# Autodesk Inventor assembly: X_rail_Assembly_Rev3
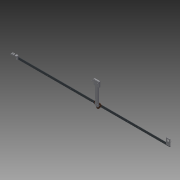
[picture p0: Inventor's stored thumbnail of the model, 180x180]
Saved by Autodesk Inventor 2015 (Build 190159000, 159)
## iProperties
Created: 2017-01-08
Part Number: X_rail_Assembly_Rev3
Document SubType Name: Assembly
Designer: Guy
Author: Guy
## Documents named in this file (12)
- C:\Users\Ernest\Documents\Capstone-Project\doc\CAD\LowLevel_Rev3\X_rail_Assembly_Rev3.iam
- C:\Users\Ernest\Documents\Capstone-Project\doc\CAD\LowLevel_Rev3\X_Rai-SquareBar-Rev3.ipt
- C:\Users\Ernest\Documents\Capstone-Project\doc\CAD\LowLevel_Rev3\XY_Wheel-SquareBar-Rev3.ipt
- C:\Users\Ernest\Documents\Capstone-Project\doc\CAD\LowLevel_Rev3\Arm-SquareBar-Rev3.ipt
- C:\Users\Ernest\Documents\Capstone-Project\doc\CAD\Nuts and Bolts\3-16in_1 1-4in_Bolt.ipt
- C:\Users\Ernest\Documents\Capstone-Project\doc\CAD\Nuts and Bolts\3-16in_7-16in_washer(num8).ipt
- C:\Users\Ernest\Documents\Capstone-Project\doc\CAD\Nuts and Bolts\3-16in_1-16in_nut(num2).ipt
- C:\Users\Ernest\Documents\Capstone-Project\doc\CAD\Stepper Motor\NEMA 23\NEMA 23 Holder.ipt
- C:\Users\Ernest\Documents\Capstone-Project\doc\CAD\LowLevel_Rev3\X_Rail_Belt_Pulley_Connector(2).ipt
- C:\Users\Ernest\Documents\Capstone-Project\doc\CAD\LowLevel_Rev3\X_Rail_Belt_Pulley_Connector.ipt
- C:\Users\Ernest\Documents\Capstone-Project\doc\CAD\LowLevel_Rev3\Arm_Base-SquareBar-Rev3-2.ipt
- C:\Users\Ernest\Documents\Capstone-Project\doc\CAD\Nuts and Bolts\L-Bracket.ipt
## Components (45 placed, 11 different names)
1. X_Rai-SquareBar-Rev3:1 — Tangent:3, Mate:3, Tangent:4, Tangent:5, Mate:88, Mate:133, Angle:2, Mate:174, Mate:175, Mate:176, Mate:177
2. XY_Wheel-SquareBar-Rev3:1 — Tangent:3, Mate:3, Flush:1, Mate:75, Mate:77, Mate:78
3. Arm-SquareBar-Rev3:1 — Mate:28, Mate:29, Mate:30, Mate:31, Mate:123, Mate:124, Mate:125, Mate:142, Mate:153, Angle:2, Mate:168, Mate:169, Mate:170, Mate:171, Mate:172, Mate:173
4. XY_Wheel-SquareBar-Rev3:2 — Tangent:4, Flush:2, Mate:68, Mate:69, Mate:118
5. XY_Wheel-SquareBar-Rev3:3 — Tangent:5, Flush:1, Flush:2, Mate:51, Mate:55, Mate:116
6. 3-16in_1 1-4in_Bolt:1 — Mate:40, Mate:41, Mate:142, Mate:156, Mate:157
7. 3-16in_7-16in_washer(num8):1 — Mate:29, Mate:32, Mate:36
8. 3-16in_7-16in_washer(num8):2 — Mate:28, Mate:33, Mate:38
9. 3-16in_7-16in_washer(num8):3 — Mate:30, Mate:35, Mate:40
10. 3-16in_7-16in_washer(num8):4 — Mate:31, Mate:34, Mate:42
11. 3-16in_1 1-4in_Bolt:2 — Mate:36, Mate:37, Mate:125, Mate:161
12. 3-16in_1 1-4in_Bolt:3 — Mate:42, Mate:43, Mate:123, Mate:154, Mate:160
13. 3-16in_1 1-4in_Bolt:4 — Mate:38, Mate:39, Mate:124, Mate:158, Mate:159
14. 3-16in_1-16in_nut(num2):1 — Mate:35, Mate:41
15. 3-16in_1-16in_nut(num2):2 — Mate:34, Mate:43, Mate:154
16. 3-16in_1-16in_nut(num2):3 — Mate:33, Mate:39
17. 3-16in_1-16in_nut(num2):4 — Mate:32, Mate:37
18. 3-16in_1 1-4in_Bolt:5 — Mate:46, Mate:48, Mate:49, Mate:52, Mate:53, Mate:116, Flush:4, Mate:146, Mate:149
19. 3-16in_1 1-4in_Bolt:6 — Mate:60, Mate:61, Mate:62, Mate:63, Mate:64, Mate:118, Mate:145, Mate:165
20. 3-16in_1 1-4in_Bolt:7 — Mate:70, Mate:71, Mate:72, Mate:73, Mate:74, Mate:75, Mate:164
21. 3-16in_1-16in_nut(num2):5 — Mate:46, Mate:148, Mate:149
22. 3-16in_1-16in_nut(num2):6 — Mate:48, Mate:50
23. 3-16in_1-16in_nut(num2):7 — Mate:53, Mate:54, Flush:4
24. 3-16in_7-16in_washer(num8):5 — Mate:49, Mate:50, Mate:55
25. 3-16in_7-16in_washer(num8):6 — Mate:51, Mate:52, Mate:54
26. 3-16in_7-16in_washer(num8):7 — Mate:56, Mate:63, Mate:69
27. 3-16in_7-16in_washer(num8):8 — Mate:57, Mate:61, Mate:68
28. 3-16in_7-16in_washer(num8):9 — Mate:58, Mate:73, Mate:78
29. 3-16in_7-16in_washer(num8):10 — Mate:59, Mate:71, Mate:77
30. 3-16in_1-16in_nut(num2):8 — Mate:56, Mate:64
31. 3-16in_1-16in_nut(num2):9 — Mate:57, Mate:62
32. 3-16in_1-16in_nut(num2):10 — Mate:60, Mate:147, Mate:165
33. 3-16in_1-16in_nut(num2):11 — Mate:58, Mate:74
34. 3-16in_1-16in_nut(num2):12 — Mate:59, Mate:72
35. 3-16in_1-16in_nut(num2):13 — Mate:70, Mate:163, Mate:164
36. NEMA 23 Holder:1 — Mate:88, Mate:106, Mate:107, Mate:141, Mate:174, Mate:175
37. XY_Wheel-SquareBar-Rev3:4 — Mate:93, Mate:140
38. 3-16in_1 1-4in_Bolt:8 — Mate:93, Mate:136, Mate:137
39. 3-16in_1 1-4in_Bolt:9 — Mate:106, Mate:107, Mate:109
40. 3-16in_1-16in_nut(num2):17 — Mate:109, Mate:141
41. X_Rail_Belt_Pulley_Connector(2):1 — Mate:136, Mate:137, Mate:138, Mate:139, Angle:1, Mate:140
42. X_Rail_Belt_Pulley_Connector:1 — Mate:133, Mate:138, Mate:139, Angle:1, Mate:176, Mate:177
43. Arm_Base-SquareBar-Rev3-2:1 — Mate:145, Mate:146, Mate:147, Mate:148, Mate:153, Mate:156, Mate:157, Mate:158, Mate:159, Mate:160, Mate:161, Mate:163
44. L-Bracket:1 — Mate:171, Mate:172, Mate:173
45. L-Bracket:2 — Mate:168, Mate:169, Mate:170
## Relationships (97: Mate 89, Tangent 3, Flush 3, Angle 2)
- Tangent:3: X_Rai-SquareBar-Rev3:1 ↔ XY_Wheel-SquareBar-Rev3:1
- Mate:3 (0.075 mm): X_Rai-SquareBar-Rev3:1 ↔ XY_Wheel-SquareBar-Rev3:1
- Tangent:4: X_Rai-SquareBar-Rev3:1 ↔ XY_Wheel-SquareBar-Rev3:2
- Tangent:5: X_Rai-SquareBar-Rev3:1 ↔ XY_Wheel-SquareBar-Rev3:3
- Flush:1: XY_Wheel-SquareBar-Rev3:1 ↔ XY_Wheel-SquareBar-Rev3:3
- Flush:2: XY_Wheel-SquareBar-Rev3:2 ↔ XY_Wheel-SquareBar-Rev3:3
- Mate:28: Arm-SquareBar-Rev3:1 ↔ 3-16in_7-16in_washer(num8):2
- Mate:29: Arm-SquareBar-Rev3:1 ↔ 3-16in_7-16in_washer(num8):1
- Mate:30: Arm-SquareBar-Rev3:1 ↔ 3-16in_7-16in_washer(num8):3
- Mate:31: Arm-SquareBar-Rev3:1 ↔ 3-16in_7-16in_washer(num8):4
- Mate:32: 3-16in_7-16in_washer(num8):1 ↔ 3-16in_1-16in_nut(num2):4
- Mate:33: 3-16in_7-16in_washer(num8):2 ↔ 3-16in_1-16in_nut(num2):3
- Mate:34: 3-16in_7-16in_washer(num8):4 ↔ 3-16in_1-16in_nut(num2):2
- Mate:35: 3-16in_7-16in_washer(num8):3 ↔ 3-16in_1-16in_nut(num2):1
- Mate:36: 3-16in_7-16in_washer(num8):1 ↔ 3-16in_1 1-4in_Bolt:2
- Mate:37: 3-16in_1 1-4in_Bolt:2 ↔ 3-16in_1-16in_nut(num2):4
- Mate:38: 3-16in_7-16in_washer(num8):2 ↔ 3-16in_1 1-4in_Bolt:4
- Mate:39: 3-16in_1 1-4in_Bolt:4 ↔ 3-16in_1-16in_nut(num2):3
- Mate:40: 3-16in_1 1-4in_Bolt:1 ↔ 3-16in_7-16in_washer(num8):3
- Mate:41: 3-16in_1 1-4in_Bolt:1 ↔ 3-16in_1-16in_nut(num2):1
- Mate:42: 3-16in_7-16in_washer(num8):4 ↔ 3-16in_1 1-4in_Bolt:3
- Mate:43: 3-16in_1 1-4in_Bolt:3 ↔ 3-16in_1-16in_nut(num2):2
- Mate:46: 3-16in_1 1-4in_Bolt:5 ↔ 3-16in_1-16in_nut(num2):5
- Mate:48: 3-16in_1 1-4in_Bolt:5 ↔ 3-16in_1-16in_nut(num2):6
- Mate:49: 3-16in_1 1-4in_Bolt:5 ↔ 3-16in_7-16in_washer(num8):5
- Mate:50: 3-16in_1-16in_nut(num2):6 ↔ 3-16in_7-16in_washer(num8):5
- Mate:51: XY_Wheel-SquareBar-Rev3:3 ↔ 3-16in_7-16in_washer(num8):6
- Mate:52: 3-16in_1 1-4in_Bolt:5 ↔ 3-16in_7-16in_washer(num8):6
- Mate:53: 3-16in_1 1-4in_Bolt:5 ↔ 3-16in_1-16in_nut(num2):7
- Mate:54: 3-16in_1-16in_nut(num2):7 ↔ 3-16in_7-16in_washer(num8):6
- Mate:55: XY_Wheel-SquareBar-Rev3:3 ↔ 3-16in_7-16in_washer(num8):5
- Mate:56: 3-16in_7-16in_washer(num8):7 ↔ 3-16in_1-16in_nut(num2):8
- Mate:57: 3-16in_7-16in_washer(num8):8 ↔ 3-16in_1-16in_nut(num2):9
- Mate:58: 3-16in_7-16in_washer(num8):9 ↔ 3-16in_1-16in_nut(num2):11
- Mate:59: 3-16in_7-16in_washer(num8):10 ↔ 3-16in_1-16in_nut(num2):12
- Mate:60: 3-16in_1 1-4in_Bolt:6 ↔ 3-16in_1-16in_nut(num2):10
- Mate:61: 3-16in_1 1-4in_Bolt:6 ↔ 3-16in_7-16in_washer(num8):8
- Mate:62: 3-16in_1 1-4in_Bolt:6 ↔ 3-16in_1-16in_nut(num2):9
- Mate:63: 3-16in_1 1-4in_Bolt:6 ↔ 3-16in_7-16in_washer(num8):7
- Mate:64: 3-16in_1 1-4in_Bolt:6 ↔ 3-16in_1-16in_nut(num2):8
- Mate:68: XY_Wheel-SquareBar-Rev3:2 ↔ 3-16in_7-16in_washer(num8):8
- Mate:69: XY_Wheel-SquareBar-Rev3:2 ↔ 3-16in_7-16in_washer(num8):7
- Mate:70: 3-16in_1 1-4in_Bolt:7 ↔ 3-16in_1-16in_nut(num2):13
- Mate:71: 3-16in_1 1-4in_Bolt:7 ↔ 3-16in_7-16in_washer(num8):10
- Mate:72: 3-16in_1 1-4in_Bolt:7 ↔ 3-16in_1-16in_nut(num2):12
- Mate:73: 3-16in_1 1-4in_Bolt:7 ↔ 3-16in_7-16in_washer(num8):9
- Mate:74: 3-16in_1 1-4in_Bolt:7 ↔ 3-16in_1-16in_nut(num2):11
- Mate:75: XY_Wheel-SquareBar-Rev3:1 ↔ 3-16in_1 1-4in_Bolt:7
- Mate:77: XY_Wheel-SquareBar-Rev3:1 ↔ 3-16in_7-16in_washer(num8):10
- Mate:78: XY_Wheel-SquareBar-Rev3:1 ↔ 3-16in_7-16in_washer(num8):9
- Mate:88: X_Rai-SquareBar-Rev3:1 ↔ NEMA 23 Holder:1
- Mate:93: XY_Wheel-SquareBar-Rev3:4 ↔ 3-16in_1 1-4in_Bolt:8
- Mate:106: NEMA 23 Holder:1 ↔ 3-16in_1 1-4in_Bolt:9
- Mate:107: NEMA 23 Holder:1 ↔ 3-16in_1 1-4in_Bolt:9
- Mate:109: 3-16in_1 1-4in_Bolt:9 ↔ 3-16in_1-16in_nut(num2):17
- Mate:116: XY_Wheel-SquareBar-Rev3:3 ↔ 3-16in_1 1-4in_Bolt:5
- Mate:118: XY_Wheel-SquareBar-Rev3:2 ↔ 3-16in_1 1-4in_Bolt:6
- Mate:123: Arm-SquareBar-Rev3:1 ↔ 3-16in_1 1-4in_Bolt:3
- Mate:124: Arm-SquareBar-Rev3:1 ↔ 3-16in_1 1-4in_Bolt:4
- Mate:125: Arm-SquareBar-Rev3:1 ↔ 3-16in_1 1-4in_Bolt:2
- Flush:4 (-3 mm): 3-16in_1 1-4in_Bolt:5 ↔ 3-16in_1-16in_nut(num2):7
- Mate:133: X_Rai-SquareBar-Rev3:1 ↔ X_Rail_Belt_Pulley_Connector:1
- Mate:136: 3-16in_1 1-4in_Bolt:8 ↔ X_Rail_Belt_Pulley_Connector(2):1
- Mate:137: 3-16in_1 1-4in_Bolt:8 ↔ X_Rail_Belt_Pulley_Connector(2):1
- Mate:138: X_Rail_Belt_Pulley_Connector(2):1 ↔ X_Rail_Belt_Pulley_Connector:1
- Mate:139 (20 mm): X_Rail_Belt_Pulley_Connector(2):1 ↔ X_Rail_Belt_Pulley_Connector:1
- Angle:1 (180 deg): X_Rail_Belt_Pulley_Connector(2):1 ↔ X_Rail_Belt_Pulley_Connector:1
- Mate:140 (6 mm): XY_Wheel-SquareBar-Rev3:4 ↔ X_Rail_Belt_Pulley_Connector(2):1
- Mate:141: NEMA 23 Holder:1 ↔ 3-16in_1-16in_nut(num2):17
- Mate:142: Arm-SquareBar-Rev3:1 ↔ 3-16in_1 1-4in_Bolt:1
- Mate:145: 3-16in_1 1-4in_Bolt:6 ↔ Arm_Base-SquareBar-Rev3-2:1
- Mate:146: 3-16in_1 1-4in_Bolt:5 ↔ Arm_Base-SquareBar-Rev3-2:1
- Mate:147: 3-16in_1-16in_nut(num2):10 ↔ Arm_Base-SquareBar-Rev3-2:1
- Mate:148: 3-16in_1-16in_nut(num2):5 ↔ Arm_Base-SquareBar-Rev3-2:1
- Mate:149: 3-16in_1 1-4in_Bolt:5 ↔ 3-16in_1-16in_nut(num2):5
- Mate:153: Arm-SquareBar-Rev3:1 ↔ Arm_Base-SquareBar-Rev3-2:1
- Mate:154: 3-16in_1 1-4in_Bolt:3 ↔ 3-16in_1-16in_nut(num2):2
- Mate:156: 3-16in_1 1-4in_Bolt:1 ↔ Arm_Base-SquareBar-Rev3-2:1
- Mate:157: 3-16in_1 1-4in_Bolt:1 ↔ Arm_Base-SquareBar-Rev3-2:1
- Mate:158: 3-16in_1 1-4in_Bolt:4 ↔ Arm_Base-SquareBar-Rev3-2:1
- Mate:159: 3-16in_1 1-4in_Bolt:4 ↔ Arm_Base-SquareBar-Rev3-2:1
- Mate:160: 3-16in_1 1-4in_Bolt:3 ↔ Arm_Base-SquareBar-Rev3-2:1
- Mate:161: 3-16in_1 1-4in_Bolt:2 ↔ Arm_Base-SquareBar-Rev3-2:1
- Mate:163: 3-16in_1-16in_nut(num2):13 ↔ Arm_Base-SquareBar-Rev3-2:1
- Mate:164: 3-16in_1 1-4in_Bolt:7 ↔ 3-16in_1-16in_nut(num2):13
- Mate:165: 3-16in_1 1-4in_Bolt:6 ↔ 3-16in_1-16in_nut(num2):10
- Angle:2 (0 deg): X_Rai-SquareBar-Rev3:1 ↔ Arm-SquareBar-Rev3:1
- Mate:168: Arm-SquareBar-Rev3:1 ↔ L-Bracket:2
- Mate:169: Arm-SquareBar-Rev3:1 ↔ L-Bracket:2
- Mate:170: Arm-SquareBar-Rev3:1 ↔ L-Bracket:2
- Mate:171: Arm-SquareBar-Rev3:1 ↔ L-Bracket:1
- Mate:172: Arm-SquareBar-Rev3:1 ↔ L-Bracket:1
- Mate:173: Arm-SquareBar-Rev3:1 ↔ L-Bracket:1
- Mate:174: X_Rai-SquareBar-Rev3:1 ↔ NEMA 23 Holder:1
- Mate:175: X_Rai-SquareBar-Rev3:1 ↔ NEMA 23 Holder:1
- Mate:176: X_Rai-SquareBar-Rev3:1 ↔ X_Rail_Belt_Pulley_Connector:1
- Mate:177: X_Rai-SquareBar-Rev3:1 ↔ X_Rail_Belt_Pulley_Connector:1
